# Autodesk Inventor assembly: パネル型スカラアーム
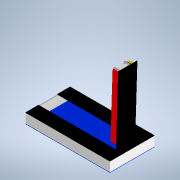
[picture p0: Inventor's stored thumbnail of the model, 180x180]
Saved by Autodesk Inventor 2022 (Build 260153000, 153)
## iProperties
Created: 2022-10-17
Part Number: パネル型スカラアーム
Document SubType Name: Assembly
Designer: tdn82
Mass: 1402.96 g
Surface Area: 5352.73 cm^2
Volume: 859.492 cm^3
Density: 1.63232 g/cm^3
Author: tdn82
## Documents named in this file (16)
- C:\Users\tdn82\OneDrive\ドキュメント\Inventor\卒業研究パネル型スカラアーム\GrabCAD\panel-type-scalar-arm\パネル型スカラアーム\パネル型スカラアーム.iam
- C:\Users\tdn82\OneDrive\ドキュメント\Inventor\卒業研究パネル型スカラアーム\GrabCAD\panel-type-scalar-arm\パネル型スカラアーム\縦長フラットバー右.ipt
- C:\Users\tdn82\OneDrive\ドキュメント\Inventor\卒業研究パネル型スカラアーム\GrabCAD\panel-type-scalar-arm\パネル型スカラアーム\横長フラットバー.ipt
- C:\Users\tdn82\OneDrive\ドキュメント\Inventor\卒業研究パネル型スカラアーム\GrabCAD\panel-type-scalar-arm\パネル型スカラアーム\サーボモータB3M-SC-1170-AB3M1100_scale.ipt
- C:\Users\tdn82\OneDrive\ドキュメント\Inventor\卒業研究パネル型スカラアーム\GrabCAD\panel-type-scalar-arm\パネル型スカラアーム\後ろカバー.ipt
- C:\Users\tdn82\OneDrive\ドキュメント\Inventor\卒業研究パネル型スカラアーム\GrabCAD\panel-type-scalar-arm\パネル型スカラアーム\横長3rdフラットバー下.ipt
- C:\Users\tdn82\OneDrive\ドキュメント\Inventor\卒業研究パネル型スカラアーム\GrabCAD\panel-type-scalar-arm\パネル型スカラアーム\縦長3rdフラットバー.ipt
- C:\Users\tdn82\OneDrive\ドキュメント\Inventor\卒業研究パネル型スカラアーム\GrabCAD\panel-type-scalar-arm\パネル型スカラアーム\１段目アーム.iam
- C:\Users\tdn82\OneDrive\ドキュメント\Inventor\卒業研究パネル型スカラアーム\GrabCAD\panel-type-scalar-arm\パネル型スカラアーム\横長2ndフラットバー下.ipt
- C:\Users\tdn82\OneDrive\ドキュメント\Inventor\卒業研究パネル型スカラアーム\GrabCAD\panel-type-scalar-arm\パネル型スカラアーム\横長3rdフラットバー上.ipt
- C:\Users\tdn82\OneDrive\ドキュメント\Inventor\卒業研究パネル型スカラアーム\GrabCAD\panel-type-scalar-arm\パネル型スカラアーム\サーボモータ固定用２軸目.ipt
- C:\Users\tdn82\OneDrive\ドキュメント\Inventor\卒業研究パネル型スカラアーム\GrabCAD\panel-type-scalar-arm\パネル型スカラアーム\前上下カバーサーボ隠し.ipt
- C:\Users\tdn82\OneDrive\ドキュメント\Inventor\卒業研究パネル型スカラアーム\GrabCAD\panel-type-scalar-arm\パネル型スカラアーム\前カバー中盤左アーム固定.ipt
- C:\Users\tdn82\OneDrive\ドキュメント\Inventor\卒業研究パネル型スカラアーム\GrabCAD\panel-type-scalar-arm\パネル型スカラアーム\前カバー中段右.ipt
- C:\Users\tdn82\OneDrive\ドキュメント\Inventor\卒業研究パネル型スカラアーム\GrabCAD\panel-type-scalar-arm\パネル型スカラアーム\サーボ固定パーツ３Dプリンタ出力実験\サーボモータ固定用２軸目5mm.ipt
- C:\Users\tdn82\OneDrive\ドキュメント\Inventor\卒業研究パネル型スカラアーム\GrabCAD\panel-type-scalar-arm\パネル型スカラアーム\サーボ固定パーツ３Dプリンタ出力実験\サーボモータ固定用２軸目4mm改.ipt
## Components (18 placed, 15 different names)
1. 縦長フラットバー右:1 — メイト:1, フラッシュ:1, フラッシュ:2, フラッシュ:3, メイト:2, メイト:3, メイト:4, メイト:12
2. 縦長フラットバー右:2 — メイト:5, メイト:6, メイト:7, メイト:8, 挿入:1, 挿入:2, メイト:22, メイト:24, メイト:29, メイト:31
3. 横長フラットバー:1 — メイト:2, メイト:3, メイト:4, メイト:5, メイト:6, メイト:11, メイト:23
4. 横長フラットバー:3 — メイト:7, メイト:8, メイト:25
5. サーボモータB3M-SC-1170-AB3M1100_scale:2 — 挿入:15, 挿入:16, 挿入:17
6. 後ろカバー:1 — メイト:11, メイト:12
7. 横長3rdフラットバー下:2 — メイト:18, メイト:19, 挿入:17
8. 縦長3rdフラットバー:1 — メイト:18, メイト:19, メイト:20, メイト:21
9. １段目アーム:1 [sub-assembly] — 挿入:1, 挿入:2, 挿入:12
10. 横長2ndフラットバー下:2 — メイト:26, メイト:27, メイト:28, 挿入:12
11. 横長3rdフラットバー上:1 — メイト:20, メイト:21
12. 前上下カバーサーボ隠し:1 — メイト:22, メイト:23, メイト:30
13. 前上下カバーサーボ隠し:2 — メイト:24, メイト:25
14. 前カバー中盤左アーム固定:1 — メイト:26, メイト:27, メイト:28, 挿入:10, 挿入:11, 挿入:13, 挿入:14, 挿入:18, 挿入:19
15. サーボモータ固定用２軸目:1 — 挿入:10, 挿入:11
16. 前カバー中段右:1 — メイト:29, メイト:30, メイト:31
17. サーボモータ固定用２軸目5mm:1 — 挿入:13, 挿入:14, 挿入:15, 挿入:16
18. サーボモータ固定用２軸目4mm改:1 — 挿入:18, 挿入:19
## Relationships (39: Mate 24, Insert 12, Flush 3)
- メイト:1 [Mate]: 縦長フラットバー右:1
- フラッシュ:1 [Flush]: 縦長フラットバー右:1
- フラッシュ:2 [Flush]: 縦長フラットバー右:1
- フラッシュ:3 [Flush]: 縦長フラットバー右:1
- メイト:2 [Mate]: 縦長フラットバー右:1 ↔ 横長フラットバー:1
- メイト:3 [Mate]: 縦長フラットバー右:1 ↔ 横長フラットバー:1
- メイト:4 [Mate]: 縦長フラットバー右:1 ↔ 横長フラットバー:1
- メイト:5 [Mate]: 縦長フラットバー右:2 ↔ 横長フラットバー:1
- メイト:6 [Mate]: 縦長フラットバー右:2 ↔ 横長フラットバー:1
- メイト:7 [Mate]: 縦長フラットバー右:2 ↔ 横長フラットバー:3
- メイト:8 [Mate]: 縦長フラットバー右:2 ↔ 横長フラットバー:3
- メイト:11 [Mate]: 横長フラットバー:1 ↔ 後ろカバー:1
- メイト:12 [Mate]: 縦長フラットバー右:1 ↔ 後ろカバー:1
- メイト:18 [Mate]: 横長3rdフラットバー下:2 ↔ 縦長3rdフラットバー:1
- メイト:19 [Mate]: 横長3rdフラットバー下:2 ↔ 縦長3rdフラットバー:1
- 挿入:1 [Insert]: 縦長フラットバー右:2 ↔ １段目アーム:1
- 挿入:2 [Insert]: 縦長フラットバー右:2 ↔ １段目アーム:1
- メイト:20 [Mate]: 縦長3rdフラットバー:1 ↔ 横長3rdフラットバー上:1
- メイト:21 [Mate]: 縦長3rdフラットバー:1 ↔ 横長3rdフラットバー上:1
- メイト:22 [Mate]: 縦長フラットバー右:2 ↔ 前上下カバーサーボ隠し:1
- メイト:23 [Mate]: 横長フラットバー:1 ↔ 前上下カバーサーボ隠し:1
- メイト:24 [Mate]: 縦長フラットバー右:2 ↔ 前上下カバーサーボ隠し:2
- メイト:25 [Mate]: 横長フラットバー:3 ↔ 前上下カバーサーボ隠し:2
- メイト:26 [Mate]: 横長2ndフラットバー下:2 ↔ 前カバー中盤左アーム固定:1
- メイト:27 [Mate] (0.5 mm): 横長2ndフラットバー下:2 ↔ 前カバー中盤左アーム固定:1
- メイト:28 [Mate] (11 mm): 横長2ndフラットバー下:2 ↔ 前カバー中盤左アーム固定:1
- 挿入:10 [Insert]: 前カバー中盤左アーム固定:1 ↔ サーボモータ固定用２軸目:1
- 挿入:11 [Insert]: 前カバー中盤左アーム固定:1 ↔ サーボモータ固定用２軸目:1
- メイト:29 [Mate]: 縦長フラットバー右:2 ↔ 前カバー中段右:1
- メイト:30 [Mate]: 前上下カバーサーボ隠し:1 ↔ 前カバー中段右:1
- メイト:31 [Mate]: 縦長フラットバー右:2 ↔ 前カバー中段右:1
- 挿入:12 [Insert]: １段目アーム:1 ↔ 横長2ndフラットバー下:2
- 挿入:13 [Insert]: 前カバー中盤左アーム固定:1 ↔ サーボモータ固定用２軸目5mm:1
- 挿入:14 [Insert]: 前カバー中盤左アーム固定:1 ↔ サーボモータ固定用２軸目5mm:1
- 挿入:15 [Insert]: サーボモータB3M-SC-1170-AB3M1100_scale:2 ↔ サーボモータ固定用２軸目5mm:1
- 挿入:16 [Insert]: サーボモータB3M-SC-1170-AB3M1100_scale:2 ↔ サーボモータ固定用２軸目5mm:1
- 挿入:17 [Insert]: サーボモータB3M-SC-1170-AB3M1100_scale:2 ↔ 横長3rdフラットバー下:2
- 挿入:18 [Insert]: 前カバー中盤左アーム固定:1 ↔ サーボモータ固定用２軸目4mm改:1
- 挿入:19 [Insert]: 前カバー中盤左アーム固定:1 ↔ サーボモータ固定用２軸目4mm改:1
